# Autodesk Inventor assembly: Tile Field
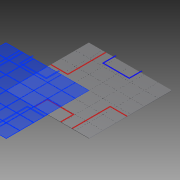
[picture p0: Inventor's stored thumbnail of the model, 180x180]
Saved by Autodesk Inventor 2015 (Build 190159000, 159)
## iProperties
Created: 2015-04-21
Part Number: Tile Field
Document SubType Name: Assembly
Designer: David Tenney
Author: David Tenney
## Documents named in this file (7)
- C:\Users\David Tenney\Documents\Inventor\Tile Field.iam
- C:\Users\David Tenney\Documents\Inventor\Corner soft tile.ipt
- C:\Users\David Tenney\Documents\Inventor\Side soft tile.ipt
- C:\Users\David Tenney\Documents\Inventor\Standard soft tile.ipt
- C:\Users\David Tenney\Documents\Inventor\Floor goal tape.ipt
- C:\Users\David Tenney\Documents\Inventor\protected zone tape.ipt
- C:\Users\David Tenney\Documents\GitHub\CAD\Field\protected zone tape Red.ipt
## Components (40 placed, 40 different names)
1. Corner soft tile_277 — Flush:32, Rigid:35
2. Corner soft tile_278 — Flush:1, Rigid:1
3. Corner soft tile_279 — Flush:27, Flush:28, Rigid:30, Rigid:31
4. Corner soft tile_280 — Flush:4, Flush:6, Rigid:5, Rigid:6
5. Side soft tile_281 — Flush:23, Rigid:24, Rigid:25
6. Side soft tile_282 — Flush:31, Flush:32, Rigid:34, Rigid:35
7. Side soft tile_283 — Flush:22, Flush:23, Rigid:23, Rigid:24, Flush:34, Flush:35, Mate:2
8. Side soft tile_284 — Flush:12, Flush:19, Rigid:12, Rigid:13
9. Side soft tile_285 — Flush:11, Flush:19, Rigid:11, Rigid:12
10. Side soft tile_286 — Flush:30, Flush:31, Rigid:33, Rigid:34
11. Side soft tile_287 — Flush:29, Flush:30, Rigid:32, Rigid:33
12. Side soft tile_288 — Flush:28, Flush:29, Rigid:31, Rigid:32
13. Side soft tile_289 — Flush:26, Flush:27, Rigid:29, Rigid:30
14. Side soft tile_290 — Flush:18, Rigid:18, Rigid:19, Flush:36, Flush:37, Mate:3
15. Side soft tile_291 — Flush:16, Rigid:17, Rigid:18
16. Side soft tile_292 — Flush:6, Flush:7, Rigid:6, Rigid:7
17. Side soft tile_293 — Flush:4, Flush:5, Rigid:4, Rigid:5
18. Side soft tile_294 — Flush:3, Flush:5, Rigid:3, Rigid:4
19. Side soft tile_295 — Flush:2, Flush:3, Rigid:2, Rigid:3, Flush:40
20. Side soft tile_296 — Flush:1, Flush:2, Rigid:1, Rigid:2, Mate:4
21. Standard soft tile_297 — Flush:24, Rigid:25, Rigid:26
22. Standard soft tile_298 — Flush:24, Flush:25, Rigid:26, Rigid:27
23. Standard soft tile_299 — Flush:25, Rigid:27, Rigid:28
24. Standard soft tile_300 — Flush:26, Rigid:28, Rigid:29
25. Standard soft tile_301 — Flush:22, Rigid:22, Rigid:23
26. Standard soft tile_302 — Flush:21, Rigid:21, Rigid:22
27. Standard soft tile_303 — Flush:20, Flush:21, Rigid:20, Rigid:21
28. Standard soft tile_304 — Flush:18, Flush:20, Rigid:19, Rigid:20
29. Standard soft tile_305 — Flush:12, Flush:13, Rigid:13, Rigid:14
30. Standard soft tile_306 — Flush:13, Flush:14, Rigid:14, Rigid:15
31. Standard soft tile_307 — Flush:14, Flush:15, Rigid:15, Rigid:16
32. Standard soft tile_308 — Flush:15, Flush:16, Rigid:16, Rigid:17
33. Standard soft tile_309 — Flush:10, Flush:11, Rigid:10, Rigid:11
34. Standard soft tile_310 — Flush:9, Flush:10, Rigid:9, Rigid:10
35. Standard soft tile_311 — Flush:8, Flush:9, Rigid:8, Rigid:9
36. Standard soft tile_312 — Flush:7, Flush:8, Rigid:7, Rigid:8
37. Floor goal tape_313 — Flush:34, Flush:35, Mate:2, Flush:39
38. Floor goal tape_314 — Flush:36, Flush:37, Mate:3
39. protected zone tape_315 — Flush:39, Flush:40, Mate:4
40. protected zone tape_316
## Relationships (75: Flush 37, WeldJoint 35, Mate 3)
- Flush:1: Corner soft tile_278 ↔ Side soft tile_296
- Flush:2: Side soft tile_295 ↔ Side soft tile_296
- Flush:3: Side soft tile_294 ↔ Side soft tile_295
- Flush:4: Corner soft tile_280 ↔ Side soft tile_293
- Flush:5: Side soft tile_293 ↔ Side soft tile_294
- Flush:6: Corner soft tile_280 ↔ Side soft tile_292
- Flush:7: Side soft tile_292 ↔ Standard soft tile_312
- Flush:8: Standard soft tile_311 ↔ Standard soft tile_312
- Flush:9: Standard soft tile_310 ↔ Standard soft tile_311
- Flush:10: Standard soft tile_309 ↔ Standard soft tile_310
- Flush:11: Side soft tile_285 ↔ Standard soft tile_309
- Flush:12: Side soft tile_284 ↔ Standard soft tile_305
- Flush:13: Standard soft tile_305 ↔ Standard soft tile_306
- Flush:14: Standard soft tile_306 ↔ Standard soft tile_307
- Flush:15: Standard soft tile_307 ↔ Standard soft tile_308
- Flush:16: Side soft tile_291 ↔ Standard soft tile_308
- Flush:18: Side soft tile_290 ↔ Standard soft tile_304
- Flush:19: Side soft tile_284 ↔ Side soft tile_285
- Flush:20: Standard soft tile_303 ↔ Standard soft tile_304
- Flush:21: Standard soft tile_302 ↔ Standard soft tile_303
- Flush:22: Side soft tile_283 ↔ Standard soft tile_301
- Flush:23: Side soft tile_281 ↔ Side soft tile_283
- Flush:24: Standard soft tile_297 ↔ Standard soft tile_298
- Flush:25: Standard soft tile_298 ↔ Standard soft tile_299
- Flush:26: Side soft tile_289 ↔ Standard soft tile_300
- Flush:27: Corner soft tile_279 ↔ Side soft tile_289
- Flush:28: Corner soft tile_279 ↔ Side soft tile_288
- Flush:29: Side soft tile_287 ↔ Side soft tile_288
- Flush:30: Side soft tile_286 ↔ Side soft tile_287
- Flush:31: Side soft tile_282 ↔ Side soft tile_286
- Flush:32: Corner soft tile_277 ↔ Side soft tile_282
- Rigid:1 [WeldJoint]: Corner soft tile_278 ↔ Side soft tile_296
- Rigid:2 [WeldJoint]: Side soft tile_295 ↔ Side soft tile_296
- Rigid:3 [WeldJoint]: Side soft tile_294 ↔ Side soft tile_295
- Rigid:4 [WeldJoint]: Side soft tile_293 ↔ Side soft tile_294
- Rigid:5 [WeldJoint]: Corner soft tile_280 ↔ Side soft tile_293
- Rigid:6 [WeldJoint]: Corner soft tile_280 ↔ Side soft tile_292
- Rigid:7 [WeldJoint]: Side soft tile_292 ↔ Standard soft tile_312
- Rigid:8 [WeldJoint]: Standard soft tile_311 ↔ Standard soft tile_312
- Rigid:9 [WeldJoint]: Standard soft tile_310 ↔ Standard soft tile_311
- Rigid:10 [WeldJoint]: Standard soft tile_309 ↔ Standard soft tile_310
- Rigid:11 [WeldJoint]: Side soft tile_285 ↔ Standard soft tile_309
- Rigid:12 [WeldJoint]: Side soft tile_284 ↔ Side soft tile_285
- Rigid:13 [WeldJoint]: Side soft tile_284 ↔ Standard soft tile_305
- Rigid:14 [WeldJoint]: Standard soft tile_305 ↔ Standard soft tile_306
- Rigid:15 [WeldJoint]: Standard soft tile_306 ↔ Standard soft tile_307
- Rigid:16 [WeldJoint]: Standard soft tile_307 ↔ Standard soft tile_308
- Rigid:17 [WeldJoint]: Side soft tile_291 ↔ Standard soft tile_308
- Rigid:18 [WeldJoint]: Side soft tile_290 ↔ Side soft tile_291
- Rigid:19 [WeldJoint]: Side soft tile_290 ↔ Standard soft tile_304
- Rigid:20 [WeldJoint]: Standard soft tile_303 ↔ Standard soft tile_304
- Rigid:21 [WeldJoint]: Standard soft tile_302 ↔ Standard soft tile_303
- Rigid:22 [WeldJoint]: Standard soft tile_301 ↔ Standard soft tile_302
- Rigid:23 [WeldJoint]: Side soft tile_283 ↔ Standard soft tile_301
- Rigid:24 [WeldJoint]: Side soft tile_281 ↔ Side soft tile_283
- Rigid:25 [WeldJoint]: Side soft tile_281 ↔ Standard soft tile_297
- Rigid:26 [WeldJoint]: Standard soft tile_297 ↔ Standard soft tile_298
- Rigid:27 [WeldJoint]: Standard soft tile_298 ↔ Standard soft tile_299
- Rigid:28 [WeldJoint]: Standard soft tile_299 ↔ Standard soft tile_300
- Rigid:29 [WeldJoint]: Side soft tile_289 ↔ Standard soft tile_300
- Rigid:30 [WeldJoint]: Corner soft tile_279 ↔ Side soft tile_289
- Rigid:31 [WeldJoint]: Corner soft tile_279 ↔ Side soft tile_288
- Rigid:32 [WeldJoint]: Side soft tile_287 ↔ Side soft tile_288
- Rigid:33 [WeldJoint]: Side soft tile_286 ↔ Side soft tile_287
- Rigid:34 [WeldJoint]: Side soft tile_282 ↔ Side soft tile_286
- Rigid:35 [WeldJoint]: Corner soft tile_277 ↔ Side soft tile_282
- Flush:34: Side soft tile_283 ↔ Floor goal tape_313
- Flush:35: Side soft tile_283 ↔ Floor goal tape_313
- Mate:2: Side soft tile_283 ↔ Floor goal tape_313
- Flush:36: Side soft tile_290 ↔ Floor goal tape_314
- Flush:37: Side soft tile_290 ↔ Floor goal tape_314
- Mate:3: Side soft tile_290 ↔ Floor goal tape_314
- Flush:39: Floor goal tape_313 ↔ protected zone tape_315
- Flush:40: Side soft tile_295 ↔ protected zone tape_315
- Mate:4: Side soft tile_296 ↔ protected zone tape_315
